# Autodesk Inventor assembly: Chamber_BauteilHaken
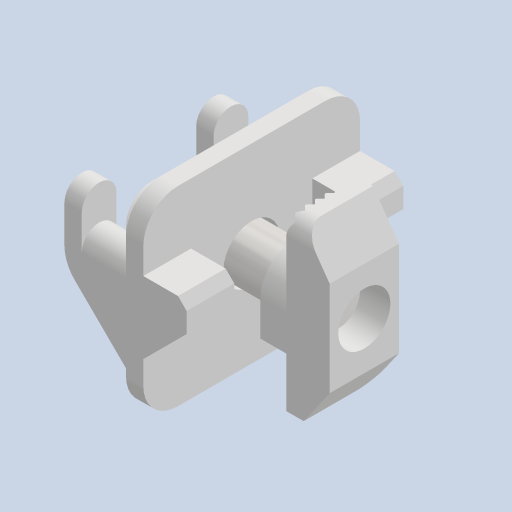
[picture p0: Inventor's stored thumbnail of the model, 512x512]
Saved by Autodesk Inventor 2023.2 (Build 272271000, 271)
## iProperties
Created: 2024-06-25
Part Number: Chamber_BauteilHaken
Document SubType Name: Assembly
Designer: Nils Bade
Author: Nils Bade
## Documents named in this file (4)
- C:\Users\nilsb\Documents\Inventor\Projektarbeit-Bade\RatRig_modified\Chamber_BauteilHaken.iam
- C:\Users\nilsb\Documents\Inventor\Projektarbeit-Bade\Schrauben\Cap Head Screw M6x12 v2.ipt
- C:\Users\nilsb\Documents\Inventor\Projektarbeit-Bade\RatRig_modified\Chamber_BauteilHaken.ipt
- C:\Users\nilsb\Documents\Inventor\Projektarbeit-Bade\RatRig_modified\T-NUT - DropIn 4040 SERIES - M6.ipt
## Components (3 placed, 3 different names)
1. Cap Head Screw M6x12 v2:1 — Passend:1, Passend:2, Passend:3
2. Chamber BauteilHaken:1 — Passend:1, Passend:2, Passend:4, Winkel:1, Fluchtend:1, Fluchtend:2
3. T-NUT - DROP IN TYPE FOR 40 SERIES - M6:1 — Passend:3, Passend:4, Winkel:1
## Relationships (7: Mate 4, Flush 2, Angle 1)
- Passend:1 [Mate]: Cap Head Screw M6x12 v2:1 ↔ Chamber BauteilHaken:1
- Passend:2 [Mate]: Cap Head Screw M6x12 v2:1 ↔ Chamber BauteilHaken:1
- Passend:3 [Mate]: Cap Head Screw M6x12 v2:1 ↔ T-NUT - DROP IN TYPE FOR 40 SERIES - M6:1
- Passend:4 [Mate] (8 mm): Chamber BauteilHaken:1 ↔ T-NUT - DROP IN TYPE FOR 40 SERIES - M6:1
- Winkel:1 [Angle] (0 deg): Chamber BauteilHaken:1 ↔ T-NUT - DROP IN TYPE FOR 40 SERIES - M6:1
- Fluchtend:1 [Flush]: Chamber BauteilHaken:1
- Fluchtend:2 [Flush]: Chamber BauteilHaken:1
